# Autodesk Inventor assembly: RFN-Setup_Vol3
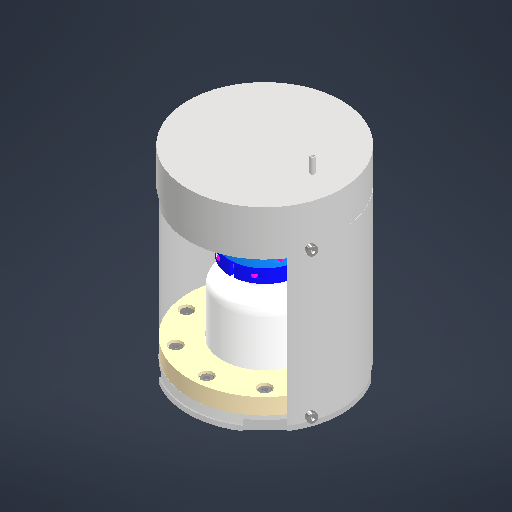
[picture p0: Inventor's stored thumbnail of the model, 512x512]
Saved by Autodesk Inventor 2027 (Build 310192060, 192F)
## iProperties
Created: 2026-07-31
Part Number: RFN-Setup_Vol3
Document SubType Name: Assembly
Designer: kw
Author: kw
## Documents named in this file (11)
- C:\Users\kw\OneDrive\Documents\Uni\Masterthesis\Spezialisierungsmodul\InventorZeichnungen_Konrad\RF-Neutralisator\RFN-Setup_Vol3.iam
- C:\Users\kw\OneDrive\Documents\Uni\Masterthesis\Spezialisierungsmodul\InventorZeichnungen_Konrad\RF-Neutralisator\Innenteil\14K_036_010_00_A_ZSB_RIM_04_3D_2016022.iam
- C:\Users\kw\OneDrive\Documents\Uni\Masterthesis\Spezialisierungsmodul\InventorZeichnungen_Konrad\RF-Neutralisator\Blende_1.ipt
- C:\Users\kw\OneDrive\Documents\Uni\Masterthesis\Spezialisierungsmodul\InventorZeichnungen_Konrad\RF-Neutralisator\GFK_Unterlegring.ipt
- C:\Users\kw\OneDrive\Documents\Uni\Masterthesis\Spezialisierungsmodul\InventorZeichnungen_Konrad\RF-Neutralisator\GFK_Ring_oben.ipt
- C:\Users\kw\OneDrive\Documents\Uni\Masterthesis\Spezialisierungsmodul\InventorZeichnungen_Konrad\RF-Neutralisator\Ring_unten.ipt
- C:\Users\kw\OneDrive\Documents\Uni\Masterthesis\Spezialisierungsmodul\InventorZeichnungen_Konrad\RF-Neutralisator\Ring_Dichtung.ipt
- C:\Users\kw\OneDrive\Documents\Uni\Masterthesis\Spezialisierungsmodul\InventorZeichnungen_Konrad\RF-Neutralisator\Abdeckung_Chamber.ipt
- C:\Users\kw\OneDrive\Documents\Uni\Masterthesis\Spezialisierungsmodul\InventorZeichnungen_Konrad\RF-Neutralisator\Abdeckung_Gaseinlass.iam
- C:\Users\kw\OneDrive\Documents\Inventor\Content Center Files\R2027\en-US\ISO 4762(2)\ISO 4762 - M3 x 10ISO.ipt
- C:\Users\kw\OneDrive\Documents\Inventor\Content Center Files\R2027\en-US\ISO 4762(2)\ISO 4762 - M4 x 12ISO.ipt
## Components (23 placed, 10 different names)
1. 14K_036_010_00_A_ZSB_RIM_04_3D_2016022:1 [sub-assembly] — Mate:3, Mate:4, Mate:8, Mate:9
2. Blende_1:1 — Mate:3, Mate:4, Mate:5
3. GFK_Unterlegring:1 — Mate:5, Mate:10, Mate:11, Mate:14
4. GFK_Ring_oben:1 — Mate:8, Mate:9, Mate:10, Mate:11, Mate:13, Mate:15, Mate:16, Insert:2
5. Ring_unten:1 — Mate:13, Mate:14, Mate:15, Mate:16, Mate:17, Mate:18, Mate:19, Mate:28, Mate:20, Mate:21, Mate:22
6. Ring_Dichtung:1 — Mate:17, Mate:18
7. Abdeckung_Chamber:1 — Mate:19, Mate:28, Mate:20, Mate:21, Mate:22, Mate:23, Mate:24, Mate:25, Mate:26, Mate:27, Insert:1
8. Abdeckung_Gaseinlass:1 [sub-assembly] — Mate:23, Mate:24, Mate:25, Mate:26, Mate:27
9. ISO 4762 M4 x 12:1 — Insert:2
10. ISO 4762 M4 x 12:2
11. ISO 4762 M4 x 12:3
12. ISO 4762 M4 x 12:4
13. ISO 4762 M4 x 12:5
14. ISO 4762 M4 x 12:6
15. ISO 4762 M4 x 12:7
16. ISO 4762 M4 x 12:8
17. ISO 4762 M4 x 12:9
18. ISO 4762 M3 x 10:1 — Insert:1
19. ISO 4762 M3 x 10:2
20. ISO 4762 M3 x 10:3
21. ISO 4762 M3 x 10:4
22. ISO 4762 M3 x 10:5
23. ISO 4762 M3 x 10:6
## Component patterns: (3 elements), (9 elements, first: ISO 4762 M4 x 12:1), (2 elements, first: ISO 4762 M3 x 10:1), Component Pattern 4:2 (2 elements), Component Pattern 4:3 (2 elements)
## Relationships (25: Mate 23, Insert 2)
- Mate:3: 14K_036_010_00_A_ZSB_RIM_04_3D_2016022:1 ↔ Blende_1:1
- Mate:4: 14K_036_010_00_A_ZSB_RIM_04_3D_2016022:1 ↔ Blende_1:1
- Mate:5: Blende_1:1 ↔ GFK_Unterlegring:1
- Mate:8: 14K_036_010_00_A_ZSB_RIM_04_3D_2016022:1 ↔ GFK_Ring_oben:1
- Mate:9: 14K_036_010_00_A_ZSB_RIM_04_3D_2016022:1 ↔ GFK_Ring_oben:1
- Mate:10: GFK_Unterlegring:1 ↔ GFK_Ring_oben:1
- Mate:11: GFK_Unterlegring:1 ↔ GFK_Ring_oben:1
- Mate:13: GFK_Ring_oben:1 ↔ Ring_unten:1
- Mate:14: GFK_Unterlegring:1 ↔ Ring_unten:1
- Mate:15: GFK_Ring_oben:1 ↔ Ring_unten:1
- Mate:16: GFK_Ring_oben:1 ↔ Ring_unten:1
- Mate:17: Ring_unten:1 ↔ Ring_Dichtung:1
- Mate:18: Ring_unten:1 ↔ Ring_Dichtung:1
- Mate:19: Ring_unten:1 ↔ Abdeckung_Chamber:1
- Mate:28: Ring_unten:1 ↔ Abdeckung_Chamber:1
- Mate:20: Ring_unten:1 ↔ Abdeckung_Chamber:1
- Mate:21: Ring_unten:1 ↔ Abdeckung_Chamber:1
- Mate:22: Ring_unten:1 ↔ Abdeckung_Chamber:1
- Mate:23: Abdeckung_Chamber:1 ↔ Abdeckung_Gaseinlass:1
- Mate:24: Abdeckung_Chamber:1 ↔ Abdeckung_Gaseinlass:1
- Mate:25: Abdeckung_Chamber:1 ↔ Abdeckung_Gaseinlass:1
- Mate:26: Abdeckung_Chamber:1 ↔ Abdeckung_Gaseinlass:1
- Mate:27: Abdeckung_Chamber:1 ↔ Abdeckung_Gaseinlass:1
- Insert:1: Abdeckung_Chamber:1 ↔ ISO 4762 M3 x 10:1
- Insert:2: GFK_Ring_oben:1 ↔ ISO 4762 M4 x 12:1
